# Autodesk Inventor assembly: roller_as,
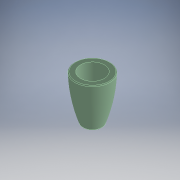
[picture p0: Inventor's stored thumbnail of the model, 180x180]
Saved by Autodesk Inventor 2022 (Build 260153000, 153)
## iProperties
Created: 2023-01-06
Part Number: roller_as,
Document SubType Name: Assembly
Designer: Иван Петров
Author: Иван Петров
## Documents named in this file (2)
- C:\Users\Ivan Petrov\Documents\GitHub\OmniBot\design\standart_components\VEX Meccanum wheel\roller_as,.iam
- C:\Users\Ivan Petrov\Documents\GitHub\OmniBot\design\standart_components\VEX Meccanum wheel\Rueda 1.ipt
## Components (1 placed, 1 different names)
1. Rueda 1:1 — Совмещение:1, Заподлицо:1
## Relationships (2: Mate 1, Flush 1)
- Совмещение:1 [Mate]: Rueda 1:1
- Заподлицо:1 [Flush]: Rueda 1:1
